# Autodesk Inventor assembly: assembly
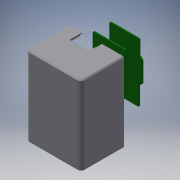
[picture p0: Inventor's stored thumbnail of the model, 180x180]
Saved by Autodesk Inventor 2018 (Build 220112000, 112)
## iProperties
Created: 2017-04-12
Part Number: assembly
Document SubType Name: Assembly
Designer: Quentin Quévy
Author: Quentin Quévy
## Documents named in this file (4)
- D:\Documents\1MAIW\MasterThesis\case\assembly.iam
- D:\Documents\1MAIW\MasterThesis\case\case.ipt
- C:\Users\Quentin Quévy\Documents\Inventor\Z1.iam
- D:\Documents\1MAIW\MasterThesis\case\Imported Components\Z1Shield\Z1Shield.iam
## Components (3 placed, 3 different names)
1. case:1 — Mate:1, Mate:2, Mate:4
2. Z1:1 [sub-assembly] — Mate:3, Flush:1
3. Z1Shield:1 [sub-assembly] — Mate:1, Mate:2, Mate:3, Flush:1, Mate:4
## Relationships (5: Mate 4, Flush 1)
- Mate:1 (10 mm): case:1 ↔ Z1Shield:1
- Mate:2 (6 mm): case:1 ↔ Z1Shield:1
- Mate:3 (15 mm): Z1:1 ↔ Z1Shield:1
- Flush:1: Z1:1 ↔ Z1Shield:1
- Mate:4: case:1 ↔ Z1Shield:1
